# Autodesk Inventor assembly: Bearing Block
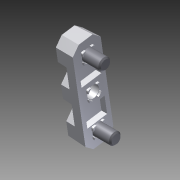
[picture p0: Inventor's stored thumbnail of the model, 180x180]
Saved by Autodesk Inventor 2014 SP1 (Build 180222100, 222)
## iProperties
Created: 2011-04-17
Part Number: Bearing Block
Document SubType Name: Assembly
Designer: Andrew
Mass: 5.39498 g
Surface Area: 21.8098 cm^2
Volume: 1.98215 cm^3
Density: 2.72178 g/cm^3
Author: Andrew
## Documents named in this file (3)
- C:\Users\Ryan\Desktop\sw\lib\Aperture VEX CAD Library\Bearing Blocks\Bearing Block with screws.iam
- C:\Users\Ryan\Desktop\sw\lib\Aperture VEX CAD Library\Hardware\8-32\8-32_.500.ipt
- C:\Users\Ryan\Desktop\sw\lib\Aperture VEX CAD Library\Bearing Blocks\Bearing Block.ipt
## Components (3 placed, 2 different names)
1. 8-32_.500:1 — Insert:2
2. Bearing Block:1 — Insert:1, Insert:2
3. 8-32_.500:2 — Insert:1
## Relationships (2: Insert 2)
- Insert:1: Bearing Block:1 ↔ 8-32_.500:2
- Insert:2: 8-32_.500:1 ↔ Bearing Block:1
